# Autodesk Inventor assembly: Transmission w 5 inch shaft and bracket assembly
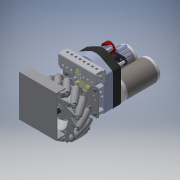
[picture p0: Inventor's stored thumbnail of the model, 180x180]
Saved by Autodesk Inventor 2016 SP2 (Build 200236200, 236)
## iProperties
Created: 2018-02-04
Part Number: Transmission w 5 inch shaft and bracket assembly
Document SubType Name: Assembly
Designer: CAD
Author: CAD
## Documents named in this file (7)
- C:\Users\CAD\Documents\GitHub\FIRST-ROBOTICS-2018-5436-CAD\Robot\Chassis\Transmission parts\Transmission w 5 inch shaft and bracket assembly.iam
- C:\Users\CAD\Desktop\new transmission layout 2.4.18.iam
- C:\Users\CAD\Downloads\217-2428-024 Rev2.ipt
- C:\Users\CAD\Documents\GitHub\FIRST-ROBOTICS-2018-5436-CAD\Robot\Chassis\wheels\am-3479R+6+SR+Mecanum+Right.iam
- C:\Users\CAD\Documents\GitHub\FIRST-ROBOTICS-2018-5436-CAD\Robot\Chassis\PVC spacers.ipt
- C:\Users\CAD\Documents\GitHub\FIRST-ROBOTICS-2018-5436-CAD\Robot\Chassis\PVC spacers 2in.ipt
- C:\Users\CAD\Documents\GitHub\FIRST-ROBOTICS-2018-5436-CAD\Robot\Chassis\shaft chassis bracket.ipt
## Components (6 placed, 6 different names)
1. new transmission layout 2.4.18:2 [sub-assembly] — Mate:1, Mate:2, Mate:3, Insert:1, Insert:2, Insert:3
2. 217-2428-024 Rev2:4 — Insert:1, Insert:2
3. am-3479R+6+SR+Mecanum+Right:1 [sub-assembly] — Mate:1, Mate:2, Mate:3
4. PVC spacers:1
5. PVC spacers 2in:1
6. shaft chassis bracket:1 — Insert:3
## Relationships (6: Mate 3, Insert 3)
- Mate:1 (38.1 mm): new transmission layout 2.4.18:2 ↔ am-3479R+6+SR+Mecanum+Right:1
- Mate:2: new transmission layout 2.4.18:2 ↔ am-3479R+6+SR+Mecanum+Right:1
- Mate:3: new transmission layout 2.4.18:2 ↔ am-3479R+6+SR+Mecanum+Right:1
- Insert:1: new transmission layout 2.4.18:2 ↔ 217-2428-024 Rev2:4
- Insert:2: new transmission layout 2.4.18:2 ↔ 217-2428-024 Rev2:4
- Insert:3: new transmission layout 2.4.18:2 ↔ shaft chassis bracket:1
